# Autodesk Inventor assembly: buttons
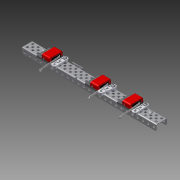
[picture p0: Inventor's stored thumbnail of the model, 180x180]
Saved by Autodesk Inventor 2014 SP1 (Build 180222100, 222)
## iProperties
Created: 2014-04-14
Part Number: buttons
Document SubType Name: Assembly
Designer: Ryan
Author: Ryan
## Documents named in this file (6)
- C:\Users\Ryan\Desktop\sw\toss up 5th A bot\tower\buttons.iam
- C:\Users\Ryan\Desktop\sw\lib\Aperture VEX CAD Library\Metal\C Channel\2 x 25.ipt
- C:\Users\Ryan\Desktop\sw\lib\Aperture VEX CAD Library\Hardware\8-32\8-23_.750.ipt
- C:\Users\Ryan\Desktop\sw\lib\Aperture VEX CAD Library\Spacers\thin\SPACER-0320-0500.ipt
- C:\Users\Ryan\Desktop\sw\toss up 5th A bot\tower\button.iam
- C:\Users\Ryan\Desktop\sw\lib\Aperture VEX CAD Library\Electronics\gyro\gyro.ipt
## Components (9 placed, 5 different names)
1. 2 x 25:1 — Mate:1, Mate:2, Mate:3, Mate:5, Mate:6, Mate:7, Mate:8, Mate:9, Mate:10, Mate:11, Mate:12, Mate:13, Mate:14, Mate:15, Mate:17, Mate:18, Mate:19, Mate:20, Mate:21
2. button:1 [sub-assembly] — Mate:6, Mate:7, Mate:8, Mate:9, Mate:10, Mate:16
3. button:2 [sub-assembly] — Mate:11, Mate:12, Mate:13, Mate:14
4. button:3 [sub-assembly] — Mate:15, Mate:16, Mate:17
5. gyro:1 — Mate:18, Mate:19, Mate:20, Mate:21
6. 8-23_.750:1 — Mate:1, Mate:2, Mate:3, Mate:4
7. SPACER-0320-0500:1 — Mate:4, Mate:5
8. 8-23_.750:2
9. SPACER-0320-0500:2
## Component patterns: (2 elements, first: 8-23_.750:1 + SPACER-0320-0500:1)
## Relationships (21: Mate 21)
- Mate:1: 2 x 25:1 ↔ 8-23_.750:1
- Mate:2 (2.3114 mm): 2 x 25:1 ↔ 8-23_.750:1
- Mate:3 (2.3114 mm): 2 x 25:1 ↔ 8-23_.750:1
- Mate:4: 8-23_.750:1 ↔ SPACER-0320-0500:1
- Mate:5: 2 x 25:1 ↔ SPACER-0320-0500:1
- Mate:6: 2 x 25:1 ↔ button:1
- Mate:7 (2.3114 mm): 2 x 25:1 ↔ button:1
- Mate:8 (2.3114 mm): 2 x 25:1 ↔ button:1
- Mate:9 (2.3114 mm): 2 x 25:1 ↔ button:1
- Mate:10 (2.3114 mm): 2 x 25:1 ↔ button:1
- Mate:11 (2.3114 mm): 2 x 25:1 ↔ button:2
- Mate:12 (15.0114 mm): 2 x 25:1 ↔ button:2
- Mate:13: 2 x 25:1 ↔ button:2
- Mate:14 (2.3114 mm): 2 x 25:1 ↔ button:2
- Mate:15: 2 x 25:1 ↔ button:3
- Mate:16: button:1 ↔ button:3
- Mate:17 (2.3114 mm): 2 x 25:1 ↔ button:3
- Mate:18: 2 x 25:1 ↔ gyro:1
- Mate:19 (2.3114 mm): 2 x 25:1 ↔ gyro:1
- Mate:20 (2.3114 mm): 2 x 25:1 ↔ gyro:1
- Mate:21 (2.3114 mm): 2 x 25:1 ↔ gyro:1
## Named parameters: q = 2.3114 mm
